# Autodesk Inventor assembly: JR3_sensor_setup_20
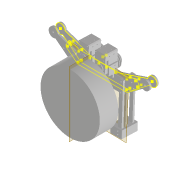
[picture p0: Inventor's stored thumbnail of the model, 180x180]
Saved by Autodesk Inventor 2022 (Build 260153000, 153)
## iProperties
Created: 2022-12-25
Part Number: JR3_sensor_setup_20
Document SubType Name: Assembly
Designer: dell
Author: dell
## Documents named in this file (3)
- D:\xxxx\Uni\Part IV\MECHENG_700\Part_IV_project_CAD\Bird_skeleton_prototypes\Wing_drone_V1\JR3_sensor_setup\JR3_sensor_setup_20.iam
- D:\xxxx\Uni\Part IV\MECHENG_700\Part_IV_project_CAD\Bird_skeleton_prototypes\Wing_drone_V1\JR3_sensor_setup\JR3_sensor.ipt
- D:\xxxx\Uni\Part IV\MECHENG_700\Part_IV_project_CAD\Bird_skeleton_prototypes\Wing_drone_V1\Bird_wing_V2\Wing_shoulder\Shoulder_support_assembly.iam
## Components (2 placed, 2 different names)
1. JR3_sensor:1 — Mate:1
2. Shoulder_support_assembly:2 [sub-assembly] — Mate:1
## Relationships (1: Mate 1)
- Mate:1: JR3_sensor:1 ↔ Shoulder_support_assembly:2
